# Autodesk Inventor assembly: 頭_1
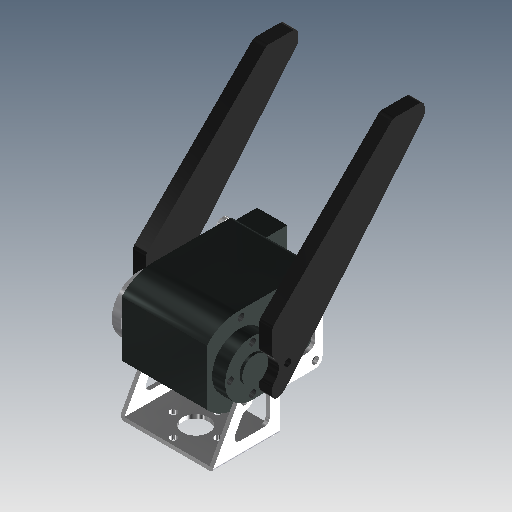
[picture p0: Inventor's stored thumbnail of the model, 512x512]
Saved by Autodesk Inventor 2017.3 (Build 213256000, 256)
## iProperties
Created: 2016-05-10
Part Number: 頭_1
Document SubType Name: Assembly
Designer: hiroaki
Mass: 109.829 g
Surface Area: 230.498 cm^2
Volume: 63.6358 cm^3
Density: 1.7259 g/cm^3
Author: hiroaki
## Documents named in this file (6)
- C:\Users\haya\Desktop\GankenKun0_5\上半身\頭\頭_1.iam
- C:\Users\haya\Desktop\GankenKun0_5\既製品\B3M10xx.ipt
- B3M11xx.ipt
- C:\Users\haya\Desktop\GankenKun0_5\上半身\頭\頭_メインフレーム_1_1.ipt
- C:\Users\haya\Desktop\GankenKun0_5\既製品\free_horn.ipt
- C:\Users\haya\Desktop\GankenKun0_5\上半身\頭\頭_サブフレーム_1_1.ipt
## Components (5 placed, 4 different names)
1. B3M11xx:1 — 挿入:3, 挿入:5, 挿入:6, メイト:6, 挿入:7, 角度:1, メイト:7
2. 頭_メインフレーム_1_1:1 — 挿入:5, 挿入:6, メイト:6
3. free_horn:1 — 挿入:3, 挿入:8
4. 頭_サブフレーム_1_1:1 — 挿入:8, メイト:7, フラッシュ:1
5. 頭_サブフレーム_1_1:2 — 挿入:7, 角度:1, フラッシュ:1
## Relationships (9: Insert 5, Mate 2, Angle 1, Flush 1)
- 挿入:3 [Insert]: B3M11xx:1 ↔ free_horn:1
- 挿入:5 [Insert]: B3M11xx:1 ↔ 頭_メインフレーム_1_1:1
- 挿入:6 [Insert]: B3M11xx:1 ↔ 頭_メインフレーム_1_1:1
- メイト:6 [Mate]: B3M11xx:1 ↔ 頭_メインフレーム_1_1:1
- 挿入:7 [Insert]: B3M11xx:1 ↔ 頭_サブフレーム_1_1:2
- 角度:1 [Angle] (0 deg): B3M11xx:1 ↔ 頭_サブフレーム_1_1:2
- 挿入:8 [Insert]: free_horn:1 ↔ 頭_サブフレーム_1_1:1
- メイト:7 [Mate]: B3M11xx:1 ↔ 頭_サブフレーム_1_1:1
- フラッシュ:1 [Flush]: 頭_サブフレーム_1_1:1 ↔ 頭_サブフレーム_1_1:2
